# Autodesk Inventor assembly: CNC_upper_skirt
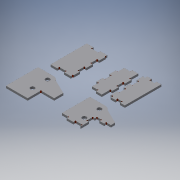
[picture p0: Inventor's stored thumbnail of the model, 180x180]
Saved by Autodesk Inventor 2016 SP2 (Build 200236200, 236)
## iProperties
Created: 2017-09-12
Part Number: CNC_upper_skirt
Document SubType Name: Assembly
Designer: Admin
Author: Admin
## Documents named in this file (6)
- E:\DATA\Inventor\AtongJali_v2\CNC_upper_skirt.iam
- E:\DATA\Inventor\AtongJali_v2\holder_base_1.ipt
- E:\DATA\Inventor\AtongJali_v2\holder_center_1.ipt
- E:\DATA\Inventor\AtongJali_v2\holder_top_1.ipt
- E:\DATA\Inventor\AtongJali_v2\side_holder_R_1.ipt
- E:\DATA\Inventor\AtongJali_v2\side_load_L_1.ipt
## Components (5 placed, 5 different names)
1. holder_base_1:1 — Flush:6
2. holder_center_1:1 — Flush:5, Flush:7
3. holder_top_1:1 — Flush:5, Flush:6, Flush:7
4. side_holder_R_1:1 — Flush:2
5. side_load_L_1:1 — Flush:2
## Relationships (4: Flush 4)
- Flush:2: side_holder_R_1:1 ↔ side_load_L_1:1
- Flush:5: holder_center_1:1 ↔ holder_top_1:1
- Flush:6: holder_base_1:1 ↔ holder_top_1:1
- Flush:7: holder_center_1:1 ↔ holder_top_1:1
